# Autodesk Inventor assembly: AM14U2_Wide
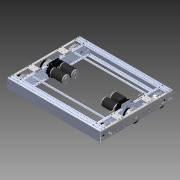
[picture p0: Inventor's stored thumbnail of the model, 180x180]
Saved by Autodesk Inventor 2015 SP1 (Build 190203100, 203)
## iProperties
Category: Drive Base
Company: Autodesk Inc.
Created: 2014-12-16
Part Number: AM14U2_Wide
Document SubType Name: Assembly
Designer: Autodesk Inc.
Catalog Web Link: andymark.com
Vendor: Andy Mark Inc.
Author: Autodesk Inc.
## Documents named in this file (2)
- D:\Data Folder\FIRST 2015\KOP_FRC\Drive Base\DB_DriveBaseWide_AM14U2.iam
- D:\Data Folder\FIRST 2015\KOP_FRC\Drive Base\Parts\AM14U2 Half Wide.iam
## Components (2 placed, 2 different names)
1. AM14U2 Half Wide_1 [sub-assembly] — Insert:1, Insert:2
2. AM14U2 Half Wide_2 [sub-assembly] — Insert:1, Insert:2
## Relationships (2: Insert 2)
- Insert:1: AM14U2 Half Wide_1 ↔ AM14U2 Half Wide_2
- Insert:2: AM14U2 Half Wide_1 ↔ AM14U2 Half Wide_2
